# Autodesk Inventor assembly: Assembly
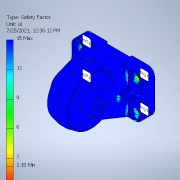
[picture p0: Inventor's stored thumbnail of the model, 180x180]
Saved by Autodesk Inventor 2020 (Build 240168000, 168)
## iProperties
Created: 2021-06-13
Part Number: Assembly
Document SubType Name: Assembly
Designer: joelm
Mass: 3418.11 g
Surface Area: 1159.77 cm^2
Volume: 475.495 cm^3
Density: 7.18853 g/cm^3
Author: joelm
## Documents named in this file (11)
- D:\Carreer 4.1\Manufacturing Tech\CAMDieSets\Assembly.iam
- D:\Carreer 4.1\Manufacturing Tech\CAMDieSets\axle.ipt
- D:\Carreer 4.1\Manufacturing Tech\CAMDieSets\axleSupport.ipt
- D:\Carreer 4.1\Manufacturing Tech\CAMDieSets\topPlate.ipt
- D:\Carreer 4.1\Manufacturing Tech\CAMDieSets\wheel.ipt
- D:\Carreer 4.1\Manufacturing Tech\CAMDieSets\Assembly\AIP\FEA\doecx1z1c.fins
- D:\Carreer 4.1\Manufacturing Tech\CAMDieSets\Assembly\AIP\FEA\doecx1z1c.fsat
- D:\Carreer 4.1\Manufacturing Tech\CAMDieSets\Assembly\AIP\FEA\doecx1z1c.ftes
- D:\Carreer 4.1\Manufacturing Tech\CAMDieSets\Assembly\AIP\FEA\doecx1z1c.fwiz
- D:\Carreer 4.1\Manufacturing Tech\CAMDieSets\Assembly\AIP\FEA\doecx1zls.fmsh
- D:\Carreer 4.1\Manufacturing Tech\CAMDieSets\Assembly\AIP\FEA\doecx1zmo.fres
## Components (5 placed, 4 different names)
1. axle:1 — Mate:1, Mate:2, Flush:1
2. axleSupport:1 — Mate:2, Flush:1, Mate:4, Mate:6, Mate:7, Flush:2
3. topPlate:1 — Mate:5, Mate:6, Mate:7, Flush:2, Flush:3
4. wheel:1 — Mate:1, Mate:3, Mate:4
5. axleSupport:2 — Mate:3, Mate:5, Flush:3
## Relationships (10: Mate 7, Flush 3)
- Mate:1: axle:1 ↔ wheel:1
- Mate:2: axle:1 ↔ axleSupport:1
- Mate:3: wheel:1 ↔ axleSupport:2
- Flush:1 (-2 mm): axle:1 ↔ axleSupport:1
- Mate:4: axleSupport:1 ↔ wheel:1
- Mate:5: topPlate:1 ↔ axleSupport:2
- Mate:6: axleSupport:1 ↔ topPlate:1
- Mate:7: axleSupport:1 ↔ topPlate:1
- Flush:2: axleSupport:1 ↔ topPlate:1
- Flush:3: topPlate:1 ↔ axleSupport:2
## Named parameters: sa_0 = 981, sa_1 = 1e+07
note: some values were not read from the file. Shown as the stored number, unit unknown: "sa_0", "sa_1".
